# Autodesk Inventor assembly: PrzekladniaLewa
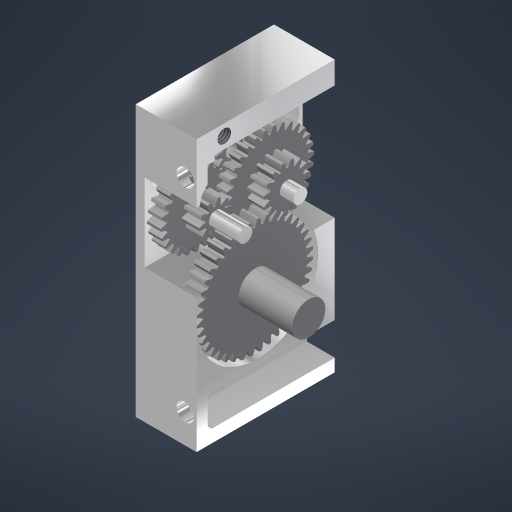
[picture p0: Inventor's stored thumbnail of the model, 512x512]
Saved by Autodesk Inventor 2023 (Build 270158000, 158)
## iProperties
Created: 2022-03-16
Part Number: PrzekladniaLewa
Material: Ogólny
Document SubType Name: Assembly
Designer: Michał
Mass: 43.9537 g
Surface Area: 113.512 cm^2
Volume: 11.9368 cm^3
Density: 3.6822 g/cm^3
Author: Michał
## Documents named in this file (8)
- D:\Projekty\RoboIlo\Ser\3D\3D\PrzekladniaLewa.iam
- D:\Projekty\RoboIlo\Ser\3D\3D\MocowanieLewejPrzekladni.ipt
- D:\Projekty\RoboIlo\Ser\3D\3D\OslonaLewejPrzekladni.ipt
- D:\Projekty\RoboIlo\Ser\3D\3D\Oś.ipt
- D:\Projekty\RoboIlo\Ser\3D\3D\PrzekladniaLewa\Design Accelerator\Przekładnie walcowe2.iam
- D:\Projekty\RoboIlo\Ser\3D\3D\PrzekladniaLewa\Design Accelerator\Przekładnie walcowe3.iam
- D:\Projekty\RoboIlo\Ser\3D\3D\PrzekladniaLewa\Design Accelerator\Przekładnie walcowe4.iam
- D:\Projekty\RoboIlo\Ser\3D\3D\Lozysko GFM-0608-06.ipt
## Components (8 placed, 5 different names)
1. MocowanieLewejPrzekladni:1 — Wstaw:1, Wstaw:3, Wstaw:4, Zestawiający:3, Wstaw:7, Zestawiający:4, Zestawiający:5, Insert:8
2. OslonaLewejPrzekladni:1 — Wstaw:1, Wstaw:7
3. Oś:1 — Wstaw:3, Zestawiający:2
4. Oś:2 — Wstaw:4, Zestawiający:1
5. Przekładnie walcowe:1 [sub-assembly] — Wstaw:5, Zestawiający:3, Zestawiający:5
6. Przekładnie walcowe:2 [sub-assembly] — Wstaw:5, Wstaw:6, Zestawiający:1
7. Przekładnie walcowe:3 [sub-assembly] — Wstaw:6, Zestawiający:2, Zestawiający:4
8. Lozysko GFM-0608-06:1 — Insert:8
## Relationships (12: Insert 7, Mate 5)
- Wstaw:1 [Insert]: MocowanieLewejPrzekladni:1 ↔ OslonaLewejPrzekladni:1
- Wstaw:3 [Insert]: MocowanieLewejPrzekladni:1 ↔ Oś:1
- Wstaw:4 [Insert]: MocowanieLewejPrzekladni:1 ↔ Oś:2
- Wstaw:5 [Insert]: Przekładnie walcowe:1 ↔ Przekładnie walcowe:2
- Wstaw:6 [Insert]: Przekładnie walcowe:2 ↔ Przekładnie walcowe:3
- Zestawiający:1 [Mate]: Oś:2 ↔ Przekładnie walcowe:2
- Zestawiający:2 [Mate]: Oś:1 ↔ Przekładnie walcowe:3
- Zestawiający:3 [Mate]: MocowanieLewejPrzekladni:1 ↔ Przekładnie walcowe:1
- Wstaw:7 [Insert]: MocowanieLewejPrzekladni:1 ↔ OslonaLewejPrzekladni:1
- Zestawiający:4 [Mate]: MocowanieLewejPrzekladni:1 ↔ Przekładnie walcowe:3
- Zestawiający:5 [Mate] (0.1 mm): MocowanieLewejPrzekladni:1 ↔ Przekładnie walcowe:1
- Insert:8: MocowanieLewejPrzekladni:1 ↔ Lozysko GFM-0608-06:1
